# Autodesk Inventor assembly: WallBody
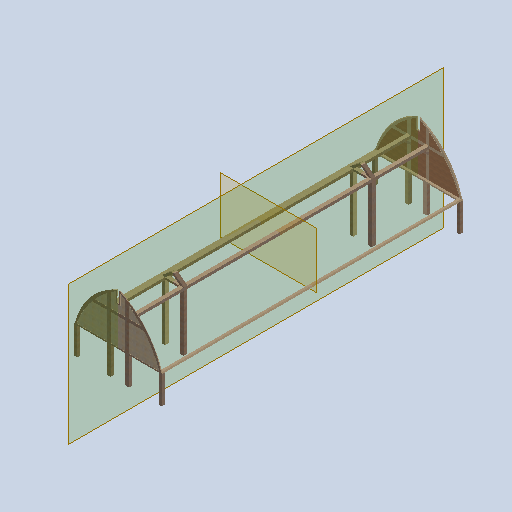
[picture p0: Inventor's stored thumbnail of the model, 512x512]
Saved by Autodesk Inventor 2024.2 (Build 282272000, 272)
## iProperties
Created: 2024-05-21
Part Number: WallBody
Document SubType Name: Assembly
Designer: LOSTER_1
Author: LOSTER_1
## Documents named in this file (44)
- C:\Users\LOSTER_1\OneDrive\桌面\school\senior\Inventor_Project\WALL\WallBody.iam
- C:\Users\LOSTER_1\OneDrive\桌面\school\senior\Inventor_Project\WALL\curve_front_wall_frame.ipt
- C:\Users\LOSTER_1\OneDrive\桌面\school\senior\Inventor_Project\WALL\top_wall_frame.ipt
- C:\Users\LOSTER_1\OneDrive\桌面\school\senior\Inventor_Project\WALL\front_wall_block01.ipt
- C:\Users\LOSTER_1\OneDrive\桌面\school\senior\Inventor_Project\WALL\front_wall_block02.ipt
- C:\Users\LOSTER_1\OneDrive\桌面\school\senior\Inventor_Project\WALL\front_wall_block03.ipt
- C:\Users\LOSTER_1\OneDrive\桌面\school\senior\Inventor_Project\WALL\front_wall_block04.ipt
- C:\Users\LOSTER_1\OneDrive\桌面\school\senior\Inventor_Project\WALL\front_wall_block01_MIR.ipt
- C:\Users\LOSTER_1\OneDrive\桌面\school\senior\Inventor_Project\WALL\front_wall_block02_MIR.ipt
- C:\Users\LOSTER_1\OneDrive\桌面\school\senior\Inventor_Project\WALL\front_wall_block03_MIR.ipt
- C:\Users\LOSTER_1\OneDrive\桌面\school\senior\Inventor_Project\WALL\front_wall_block04_MIR.ipt
- C:\Users\LOSTER_1\OneDrive\桌面\school\senior\Inventor_Project\WALL\curve_front_wall_frame_MIR.ipt
- C:\Users\LOSTER_1\OneDrive\桌面\school\senior\Inventor_Project\WALL\front_wall_block01_MIR1.ipt
- C:\Users\LOSTER_1\OneDrive\桌面\school\senior\Inventor_Project\WALL\front_wall_block02_MIR1.ipt
- C:\Users\LOSTER_1\OneDrive\桌面\school\senior\Inventor_Project\WALL\front_wall_block03_MIR1.ipt
- C:\Users\LOSTER_1\OneDrive\桌面\school\senior\Inventor_Project\WALL\front_wall_block04_MIR1.ipt
- C:\Users\LOSTER_1\OneDrive\桌面\school\senior\Inventor_Project\WALL\front_wall_block01_MIR_MIR.ipt
- C:\Users\LOSTER_1\OneDrive\桌面\school\senior\Inventor_Project\WALL\front_wall_block02_MIR_MIR.ipt
- C:\Users\LOSTER_1\OneDrive\桌面\school\senior\Inventor_Project\WALL\front_wall_block03_MIR_MIR.ipt
- C:\Users\LOSTER_1\OneDrive\桌面\school\senior\Inventor_Project\WALL\front_wall_block04_MIR_MIR.ipt
- C:\Users\LOSTER_1\OneDrive\桌面\school\senior\Inventor_Project\WALL\support_frame_01.ipt
- C:\Users\LOSTER_1\OneDrive\桌面\school\senior\Inventor_Project\WALL\support_frame_02.ipt
- C:\Users\LOSTER_1\OneDrive\桌面\school\senior\Inventor_Project\WALL\support_frame_02_MIR.ipt
- C:\Users\LOSTER_1\OneDrive\桌面\school\senior\Inventor_Project\WALL\support_frame_01_MIR.ipt
- C:\Users\LOSTER_1\OneDrive\桌面\school\senior\Inventor_Project\WALL\support_column_01.ipt
- C:\Users\LOSTER_1\OneDrive\桌面\school\senior\Inventor_Project\WALL\support_column_01_MIR.ipt
- C:\Users\LOSTER_1\OneDrive\桌面\school\senior\Inventor_Project\WALL\support_column_01_MIR1.ipt
- C:\Users\LOSTER_1\OneDrive\桌面\school\senior\Inventor_Project\WALL\support_column_01_MIR_MIR.ipt
- C:\Users\LOSTER_1\OneDrive\桌面\school\senior\Inventor_Project\WALL\support_column_02.ipt
- C:\Users\LOSTER_1\OneDrive\桌面\school\senior\Inventor_Project\WALL\support_column_02_MIR.ipt
- C:\Users\LOSTER_1\OneDrive\桌面\school\senior\Inventor_Project\WALL\support_column_02_MIR1.ipt
- C:\Users\LOSTER_1\OneDrive\桌面\school\senior\Inventor_Project\WALL\support_column_02_MIR_MIR.ipt
- C:\Users\LOSTER_1\OneDrive\桌面\school\senior\Inventor_Project\WALL\ribs\frame_rib_01.ipt
- C:\Users\LOSTER_1\OneDrive\桌面\school\senior\Inventor_Project\WALL\ribs\frame_rib_01_MIR.ipt
- C:\Users\LOSTER_1\OneDrive\桌面\school\senior\Inventor_Project\WALL\ribs\frame_rib_01_MIR1.ipt
- C:\Users\LOSTER_1\OneDrive\桌面\school\senior\Inventor_Project\WALL\ribs\frame_rib_01_MIR_MIR.ipt
- C:\Users\LOSTER_1\OneDrive\桌面\school\senior\Inventor_Project\WALL\ribs\frame_rib_02.ipt
- C:\Users\LOSTER_1\OneDrive\桌面\school\senior\Inventor_Project\WALL\ribs\frame_rib_02_MIR.ipt
- C:\Users\LOSTER_1\OneDrive\桌面\school\senior\Inventor_Project\WALL\ribs\frame_rib_02_MIR1.ipt
- C:\Users\LOSTER_1\OneDrive\桌面\school\senior\Inventor_Project\WALL\ribs\frame_rib_02_MIR_MIR.ipt
- C:\Users\LOSTER_1\OneDrive\桌面\school\senior\Inventor_Project\WALL\support_frame_03.ipt
- C:\Users\LOSTER_1\OneDrive\桌面\school\senior\Inventor_Project\WALL\support_frame_03_MIR.ipt
- C:\Users\LOSTER_1\OneDrive\桌面\school\senior\Inventor_Project\WALL\support_frame_03_MIR1.ipt
- C:\Users\LOSTER_1\OneDrive\桌面\school\senior\Inventor_Project\WALL\support_frame_03_MIR_MIR.ipt
## Components (43 placed, 43 different names)
1. curve_front_wall_frame:1 — Flush:1, Mate:1, Mate:2, Flush:2, Mate:3, Mate:4, Mate:5, Mate:7, Mate:8, Mate:9, Mate:18
2. top_wall_frame:1 — Mate:1, Mate:2, Mate:6, Mate:10, Mate:24
3. front_wall_block01:1 — Mate:3, Mate:4
4. front_wall_block02:1 — Mate:5, Mate:6
5. front_wall_block03:1 — Mate:7, Mate:8
6. front_wall_block04:1 — Mate:9, Mate:10
7. front_wall_block01_MIR:1
8. front_wall_block02_MIR:1 — Mate:19, Mate:20
9. front_wall_block03_MIR:1
10. front_wall_block04_MIR:1
11. curve_front_wall_frame_MIR:1 — Mate:11, Mate:12, Mate:13, Mate:14, Mate:15, Mate:16, Mate:17, Mate:25, Mate:26, Mate:27, Mate:28
12. front_wall_block01_MIR1:1 — Mate:12, Mate:13
13. front_wall_block02_MIR1:1 — Mate:14
14. front_wall_block03_MIR1:1 — Mate:15, Mate:16
15. front_wall_block04_MIR1:1 — Mate:17
16. front_wall_block01_MIR_MIR:1
17. front_wall_block02_MIR_MIR:1
18. front_wall_block03_MIR_MIR:1
19. front_wall_block04_MIR_MIR:1
20. support_frame_01:1 — Mate:18, Mate:19, Mate:20, Mate:21, Mate:22, Mate:23
21. support_frame_02:1 — Mate:21, Mate:22, Mate:23
22. support_frame_02_MIR:1
23. support_frame_01_MIR:1 — Mate:29, Mate:30, Mate:31, Mate:32, Mate:33, Mate:34
24. support_column_01:1 — Mate:24, Mate:25, Mate:26
25. support_column_01_MIR:1
26. support_column_01_MIR1:1
27. support_column_01_MIR_MIR:1
28. support_column_02:1 — Mate:27, Mate:28
29. support_column_02_MIR:1
30. support_column_02_MIR1:1
31. support_column_02_MIR_MIR:1
32. frame_rib_01:1 — Mate:29, Mate:30
33. frame_rib_01_MIR:1
34. frame_rib_01_MIR1:1
35. frame_rib_01_MIR_MIR:1
36. frame_rib_02:1 — Mate:31, Mate:32
37. frame_rib_02_MIR:1
38. frame_rib_02_MIR1:1
39. frame_rib_02_MIR_MIR:1
40. support_frame_03:1 — Mate:33, Mate:34
41. support_frame_03_MIR:1
42. support_frame_03_MIR1:1
43. support_frame_03_MIR_MIR:1
## Relationships (36: Mate 34, Flush 2)
- Flush:1 (16151 mm): curve_front_wall_frame:1
- Mate:1: curve_front_wall_frame:1 ↔ top_wall_frame:1
- Mate:2: curve_front_wall_frame:1 ↔ top_wall_frame:1
- Flush:2 (150 mm): curve_front_wall_frame:1
- Mate:3: curve_front_wall_frame:1 ↔ front_wall_block01:1
- Mate:4: curve_front_wall_frame:1 ↔ front_wall_block01:1
- Mate:5: curve_front_wall_frame:1 ↔ front_wall_block02:1
- Mate:6: top_wall_frame:1 ↔ front_wall_block02:1
- Mate:7: curve_front_wall_frame:1 ↔ front_wall_block03:1
- Mate:8: curve_front_wall_frame:1 ↔ front_wall_block03:1
- Mate:9: curve_front_wall_frame:1 ↔ front_wall_block04:1
- Mate:10: top_wall_frame:1 ↔ front_wall_block04:1
- Mate:11 (16151 mm): curve_front_wall_frame_MIR:1
- Mate:12: curve_front_wall_frame_MIR:1 ↔ front_wall_block01_MIR1:1
- Mate:13: curve_front_wall_frame_MIR:1 ↔ front_wall_block01_MIR1:1
- Mate:14: curve_front_wall_frame_MIR:1 ↔ front_wall_block02_MIR1:1
- Mate:15: curve_front_wall_frame_MIR:1 ↔ front_wall_block03_MIR1:1
- Mate:16: curve_front_wall_frame_MIR:1 ↔ front_wall_block03_MIR1:1
- Mate:17: curve_front_wall_frame_MIR:1 ↔ front_wall_block04_MIR1:1
- Mate:18: curve_front_wall_frame:1 ↔ support_frame_01:1
- Mate:19: front_wall_block02_MIR:1 ↔ support_frame_01:1
- Mate:20: front_wall_block02_MIR:1 ↔ support_frame_01:1
- Mate:21: support_frame_01:1 ↔ support_frame_02:1
- Mate:22: support_frame_01:1 ↔ support_frame_02:1
- Mate:23: support_frame_01:1 ↔ support_frame_02:1
- Mate:24: top_wall_frame:1 ↔ support_column_01:1
- Mate:25: curve_front_wall_frame_MIR:1 ↔ support_column_01:1
- Mate:26: curve_front_wall_frame_MIR:1 ↔ support_column_01:1
- Mate:27: curve_front_wall_frame_MIR:1 ↔ support_column_02:1
- Mate:28: curve_front_wall_frame_MIR:1 ↔ support_column_02:1
- Mate:29: support_frame_01_MIR:1 ↔ frame_rib_01:1
- Mate:30: support_frame_01_MIR:1 ↔ frame_rib_01:1
- Mate:31: support_frame_01_MIR:1 ↔ frame_rib_02:1
- Mate:32: support_frame_01_MIR:1 ↔ frame_rib_02:1
- Mate:33: support_frame_01_MIR:1 ↔ support_frame_03:1
- Mate:34: support_frame_01_MIR:1 ↔ support_frame_03:1
